# Autodesk Inventor assembly: Zespół1
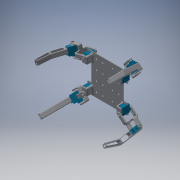
[picture p0: Inventor's stored thumbnail of the model, 180x180]
Saved by Autodesk Inventor 2018 (Build 220112000, 112)
## iProperties
Created: 2020-10-02
Part Number: Zespół1
Material: Ogólny
Document SubType Name: Assembly
Designer: Raven
Author: Raven
## Documents named in this file (6)
- C:\Users\Raven\Documents\Inventor\Pieszczoch\Zespół1.iam
- C:\Users\Raven\Documents\Inventor\Pieszczoch\noga.ipt
- C:\Users\Raven\Documents\Inventor\Pieszczoch\SG92r.ipt
- C:\Users\Raven\Documents\Inventor\Pieszczoch\orczyk_1_2.ipt
- C:\Users\Raven\Documents\Inventor\Pieszczoch\noga_2.ipt
- C:\Users\Raven\Documents\Inventor\Pieszczoch\kadlub.ipt
## Components (25 placed, 5 different names)
1. kadlub:1 — Zestawiający:13, Zestawiający:14, Równoległy:2, Zestawiający:15, Zestawiający:16, Równoległy:3, Zestawiający:17, Zestawiający:18, Równoległy:4, Zestawiający:19, Zestawiający:20, Równoległy:5
2. noga:1 — Zestawiający:1, Zestawiający:12, Równoległy:1
3. SG92r:1 — Zestawiający:1, Zestawiający:4, Zestawiający:11, Zestawiający:12, Równoległy:1
4. orczyk_1_2:1 — Zestawiający:4, Zestawiający:5, Zestawiający:6
5. noga_2:1 — Zestawiający:5, Zestawiający:8, Zestawiający:9, Zestawiający:6, Zestawiający:11
6. SG92r:2 — Zestawiający:7, Zestawiający:10, Zestawiający:13, Zestawiający:14, Równoległy:2
7. orczyk_1_2:2 — Zestawiający:7, Zestawiający:8, Zestawiający:9, Zestawiający:10
8. noga:2 — Zestawiający:46, Zestawiający:47, Równoległy:6
9. SG92r:3 — Zestawiający:46, Zestawiający:47, Zestawiający:49, Równoległy:6, Zestawiający:51
10. orczyk_1_2:3 — Zestawiający:49, Zestawiający:50, Zestawiający:51, Zestawiający:52
11. noga_2:2 — Zestawiający:50, Zestawiający:44, Zestawiający:48, Zestawiający:52
12. SG92r:8 — Zestawiający:19, Zestawiający:20, Równoległy:5, Zestawiający:42, Zestawiający:43
13. orczyk_1_2:8 — Zestawiający:42, Zestawiający:44, Zestawiający:43, Zestawiający:48
14. noga:3 — Zestawiający:39, Zestawiający:40, Zestawiający:41
15. SG92r:7 — Zestawiający:39, Zestawiający:40, Zestawiający:41, Zestawiający:57, Zestawiający:58
16. orczyk_1_2:7 — Zestawiający:57, Zestawiający:58, Zestawiający:59, Zestawiający:60
17. noga_2:4 — Zestawiający:55, Zestawiający:56, Zestawiający:59, Zestawiający:60
18. SG92r:5 — Zestawiający:15, Zestawiający:16, Równoległy:3, Zestawiający:53, Zestawiający:54
19. orczyk_1_2:5 — Zestawiający:53, Zestawiający:54, Zestawiający:55, Zestawiający:56
20. noga:4 — Zestawiający:32, Zestawiający:33, Zestawiający:34
21. SG92r:6 — Zestawiający:32, Zestawiający:33, Zestawiający:34, Zestawiający:65, Zestawiający:66
22. orczyk_1_2:6 — Zestawiający:65, Zestawiający:66, Zestawiający:67, Zestawiający:68
23. noga_2:3 — Zestawiający:63, Zestawiający:64, Zestawiający:67, Zestawiający:68
24. SG92r:4 — Zestawiający:17, Zestawiający:18, Równoległy:4, Zestawiający:61, Zestawiający:62
25. orczyk_1_2:4 — Zestawiający:61, Zestawiający:62, Zestawiający:63, Zestawiający:64
## Relationships (56: Mate 50, Flush 6)
- Zestawiający:1 [Mate]: noga:1 ↔ SG92r:1
- Zestawiający:4 [Mate]: SG92r:1 ↔ orczyk_1_2:1
- Zestawiający:5 [Mate]: orczyk_1_2:1 ↔ noga_2:1
- Zestawiający:7 [Mate]: SG92r:2 ↔ orczyk_1_2:2
- Zestawiający:8 [Mate]: noga_2:1 ↔ orczyk_1_2:2
- Zestawiający:9 [Mate]: noga_2:1 ↔ orczyk_1_2:2
- Zestawiający:6 [Mate]: orczyk_1_2:1 ↔ noga_2:1
- Zestawiający:10 [Mate]: SG92r:2 ↔ orczyk_1_2:2
- Zestawiający:11 [Mate]: SG92r:1 ↔ noga_2:1
- Zestawiający:12 [Mate]: noga:1 ↔ SG92r:1
- Równoległy:1 [Flush]: noga:1 ↔ SG92r:1
- Zestawiający:13 [Mate]: kadlub:1 ↔ SG92r:2
- Zestawiający:14 [Mate]: kadlub:1 ↔ SG92r:2
- Równoległy:2 [Flush]: kadlub:1 ↔ SG92r:2
- Zestawiający:15 [Mate]: kadlub:1 ↔ SG92r:5
- Zestawiający:16 [Mate]: kadlub:1 ↔ SG92r:5
- Równoległy:3 [Flush]: kadlub:1 ↔ SG92r:5
- Zestawiający:17 [Mate]: kadlub:1 ↔ SG92r:4
- Zestawiający:18 [Mate]: kadlub:1 ↔ SG92r:4
- Równoległy:4 [Flush]: kadlub:1 ↔ SG92r:4
- Zestawiający:19 [Mate]: kadlub:1 ↔ SG92r:8
- Zestawiający:20 [Mate]: kadlub:1 ↔ SG92r:8
- Równoległy:5 [Flush]: kadlub:1 ↔ SG92r:8
- Zestawiający:32 [Mate]: noga:4 ↔ SG92r:6
- Zestawiający:33 [Mate]: noga:4 ↔ SG92r:6
- Zestawiający:34 [Mate]: noga:4 ↔ SG92r:6
- Zestawiający:39 [Mate]: noga:3 ↔ SG92r:7
- Zestawiający:40 [Mate]: noga:3 ↔ SG92r:7
- Zestawiający:41 [Mate]: noga:3 ↔ SG92r:7
- Zestawiający:42 [Mate]: SG92r:8 ↔ orczyk_1_2:8
- Zestawiający:50 [Mate]: orczyk_1_2:3 ↔ noga_2:2
- Zestawiający:44 [Mate]: noga_2:2 ↔ orczyk_1_2:8
- Zestawiający:43 [Mate]: SG92r:8 ↔ orczyk_1_2:8
- Zestawiający:46 [Mate]: noga:2 ↔ SG92r:3
- Zestawiający:47 [Mate]: noga:2 ↔ SG92r:3
- Zestawiający:48 [Mate]: noga_2:2 ↔ orczyk_1_2:8
- Zestawiający:49 [Mate]: SG92r:3 ↔ orczyk_1_2:3
- Równoległy:6 [Flush]: noga:2 ↔ SG92r:3
- Zestawiający:51 [Mate]: SG92r:3 ↔ orczyk_1_2:3
- Zestawiający:52 [Mate]: orczyk_1_2:3 ↔ noga_2:2
- Zestawiający:53 [Mate]: SG92r:5 ↔ orczyk_1_2:5
- Zestawiający:54 [Mate]: SG92r:5 ↔ orczyk_1_2:5
- Zestawiający:55 [Mate]: noga_2:4 ↔ orczyk_1_2:5
- Zestawiający:56 [Mate]: noga_2:4 ↔ orczyk_1_2:5
- Zestawiający:57 [Mate]: SG92r:7 ↔ orczyk_1_2:7
- Zestawiający:58 [Mate]: SG92r:7 ↔ orczyk_1_2:7
- Zestawiający:59 [Mate]: orczyk_1_2:7 ↔ noga_2:4
- Zestawiający:60 [Mate]: orczyk_1_2:7 ↔ noga_2:4
- Zestawiający:61 [Mate]: SG92r:4 ↔ orczyk_1_2:4
- Zestawiający:62 [Mate]: SG92r:4 ↔ orczyk_1_2:4
- Zestawiający:63 [Mate]: noga_2:3 ↔ orczyk_1_2:4
- Zestawiający:64 [Mate]: noga_2:3 ↔ orczyk_1_2:4
- Zestawiający:65 [Mate]: SG92r:6 ↔ orczyk_1_2:6
- Zestawiający:66 [Mate]: SG92r:6 ↔ orczyk_1_2:6
- Zestawiający:67 [Mate]: orczyk_1_2:6 ↔ noga_2:3
- Zestawiający:68 [Mate]: orczyk_1_2:6 ↔ noga_2:3
